# Autodesk Inventor assembly: Remote Assembly
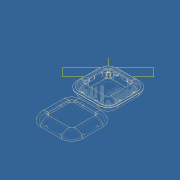
[picture p0: Inventor's stored thumbnail of the model, 180x180]
Saved by Autodesk Inventor 2,016 (Build 200138000, 138)
## iProperties
Created: 2015-06-16
Part Number: Remote Assembly
Document SubType Name: Assembly
Designer: Samuel Clay
Author: Samuel Clay
## Documents named in this file (8)
- Z:\remote\enclosure\inventor\Remote Assembly.iam
- Z:\remote\enclosure\inventor\Remote Top.ipt
- Z:\remote\enclosure\inventor\Remote Bottom.ipt
- Z:\remote\enclosure\inventor\Remote Buttons.ipt
- Z:\remote\enclosure\inventor\Remote Buttons Export.ipt
- Z:\remote\enclosure\inventor\Eagle PCB rev 21.ipt
- Z:\remote\enclosure\inventor\Case Bottom.ipt
- Z:\remote\enclosure\inventor\Case Top.ipt
## Components (7 placed, 7 different names)
1. Remote Top:1 — Flush:1
2. Remote Bottom:1
3. Remote Buttons:1 — Flush:1
4. Remote Buttons Export:1
5. Eagle PCB rev 21:1
6. Case Bottom:1
7. Case Top:1
## Relationships (1: Flush 1)
- Flush:1: Remote Top:1 ↔ Remote Buttons:1
